# Autodesk Inventor assembly: FrontWheelAssembly
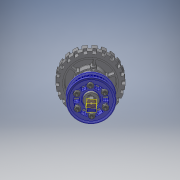
[picture p0: Inventor's stored thumbnail of the model, 180x180]
Saved by Autodesk Inventor 2016 (Build 200138000, 138)
## iProperties
Created: 2017-01-09
Part Number: FrontWheelAssembly
Document SubType Name: Assembly
Designer: Dhruv
Author: Dhruv
## Documents named in this file (8)
- C:\Users\Dhruv\Desktop\MISC\FRC 2017\supporting_parts\FrontWheelAssembly.iam
- C:\Users\Dhruv\Desktop\MISC\FRC 2017\WheelWithHexHub.iam
- C:\Users\Dhruv\Desktop\MISC\FRC 2017\Pulley.iam
- C:\Users\Dhruv\Desktop\MISC\FRC 2017\supporting_parts\217-3875-STEP-20140818.ipt
- C:\Users\Dhruv\Desktop\MISC\FRC 2017\supporting_parts\217-4002-STEP-20140806.ipt
- C:\Users\Dhruv\Desktop\MISC\FRC 2017\supporting_parts\97633A200_BLACK-FINISH STEEL EXTERNAL RETAINING RING.ipt
- C:\Users\Dhruv\Desktop\MISC\FRC 2017\supporting_parts\217-3443-STEP.ipt
- C:\Users\Dhruv\Desktop\MISC\FRC 2017\supporting_parts\217-3256-STEP.ipt
## Components (10 placed, 7 different names)
1. WheelWithHexHub:1 [sub-assembly]
2. Pulley:1 [sub-assembly]
3. 217-3875-STEP-20140818:1
4. 217-3875-STEP-20140818:2
5. 217-4002-STEP-20140806:1
6. 97633A200_BLACK-FINISH STEEL EXTERNAL RETAINING RING:1
7. 217-3443-STEP:1
8. 97633A200_BLACK-FINISH STEEL EXTERNAL RETAINING RING:2
9. 217-3256-STEP:1
10. 97633A200_BLACK-FINISH STEEL EXTERNAL RETAINING RING:3
## Relationships (23: Mate 15, RelateRotation 6, Flush 1, Insert 1)
- [Mate]: 217-3875-STEP-20140818:1 ↔ 217-4002-STEP-20140806:1
- [RelateRotation] (1 ul): 217-3875-STEP-20140818:1 ↔ 217-3875-STEP-20140818:2
- [Flush]: 217-3875-STEP-20140818:1 ↔ 217-3875-STEP-20140818:2
- [RelateRotation] (1 ul): 217-3875-STEP-20140818:2 ↔ 217-4002-STEP-20140806:1
- [Mate]: WheelWithHexHub:1 ↔ 217-4002-STEP-20140806:1
- [RelateRotation] (1 ul): WheelWithHexHub:1 ↔ 217-4002-STEP-20140806:1
- [Insert] (-25.4 mm): WheelWithHexHub:1 ↔ 217-4002-STEP-20140806:1
- [Mate]: 217-4002-STEP-20140806:1 ↔ 97633A200_BLACK-FINISH STEEL EXTERNAL RETAINING RING:1
- [Mate]: WheelWithHexHub:1 ↔ 97633A200_BLACK-FINISH STEEL EXTERNAL RETAINING RING:1
- [RelateRotation] (1 ul): 217-4002-STEP-20140806:1 ↔ 217-3443-STEP:1
- [Mate]: 217-4002-STEP-20140806:1 ↔ 217-3443-STEP:1
- [Mate]: WheelWithHexHub:1 ↔ 217-3443-STEP:1
- [Mate]: 217-4002-STEP-20140806:1 ↔ 97633A200_BLACK-FINISH STEEL EXTERNAL RETAINING RING:2
- [Mate]: 217-3443-STEP:1 ↔ 97633A200_BLACK-FINISH STEEL EXTERNAL RETAINING RING:2
- [Mate]: 217-3875-STEP-20140818:2 ↔ 97633A200_BLACK-FINISH STEEL EXTERNAL RETAINING RING:2
- [Mate]: Pulley:1 ↔ 217-4002-STEP-20140806:1
- [RelateRotation] (1 ul): Pulley:1 ↔ 217-4002-STEP-20140806:1
- [RelateRotation] (3.113 ul): 217-4002-STEP-20140806:1 ↔ 217-3256-STEP:1
- [Mate]: 217-4002-STEP-20140806:1 ↔ 217-3256-STEP:1
- [Mate]: 217-3875-STEP-20140818:1 ↔ 217-3256-STEP:1
- [Mate]: Pulley:1 ↔ 217-3256-STEP:1
- [Mate]: 217-4002-STEP-20140806:1 ↔ 97633A200_BLACK-FINISH STEEL EXTERNAL RETAINING RING:3
- [Mate]: Pulley:1 ↔ 97633A200_BLACK-FINISH STEEL EXTERNAL RETAINING RING:3
